# Autodesk Inventor assembly: comp convey
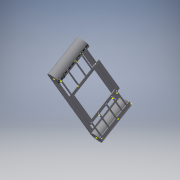
[picture p0: Inventor's stored thumbnail of the model, 180x180]
Saved by Autodesk Inventor 2019 (Build 230136000, 136)
## iProperties
Created: 2020-02-27
Part Number: comp convey
Document SubType Name: Assembly
Designer: LENOVO
Author: LENOVO
## Documents named in this file (5)
- C:\Users\LENOVO\Desktop\Abhishek\comp convey.iam
- C:\Users\LENOVO\Desktop\Abhishek\conv.ipt
- C:\Users\LENOVO\Desktop\Abhishek\connector rod.ipt
- C:\Users\LENOVO\Desktop\Abhishek\connector.ipt
- C:\Users\LENOVO\Desktop\Abhishek\roll.ipt
## Components (34 placed, 4 different names)
1. conv:1 — Mate:3, Mate:8, Mate:11, Mate:14, Mate:15, Mate:17, Mate:18, Mate:19, Mate:24, Mate:25, Mate:30, Mate:31, Mate:36, Mate:37, Mate:38, Mate:39, Mate:40, Mate:49, Mate:50, Mate:51, Mate:52, Mate:53, Mate:54, Mate:55, Mate:56, Mate:57, Mate:58, Mate:59, Mate:60, Mate:61, Mate:62, Mate:63, Mate:64, Mate:65, Mate:66, Mate:81, Mate:83, Mate:84, Mate:85, Mate:86
2. connector rod:1 — Mate:18, Mate:19, Mate:20, Mate:21, Mate:22, Mate:23
3. connector rod:2 — Mate:11, Mate:12, Mate:13, Mate:16
4. connector rod:3 — Mate:24, Mate:25, Mate:26, Mate:27, Mate:28, Mate:29
5. connector rod:5 — Mate:2, Mate:4, Mate:5, Mate:6, Mate:7, Mate:9, Mate:10
6. connector rod:6 — Mate:70, Mate:71, Mate:79
7. connector rod:7 — Mate:72, Mate:73, Mate:77
8. connector rod:8 — Mate:69, Mate:78, Mate:82
9. connector rod:10 — Mate:30, Mate:31, Mate:32, Mate:33, Mate:34, Mate:35
10. connector:1 — Mate:6, Mate:7
11. connector:3 — Mate:9, Mate:10, Mate:17
12. connector:4 — Mate:12, Mate:13, Mate:14
13. connector:7 — Mate:15, Mate:16
14. connector:8 — Mate:26, Mate:29
15. connector:9 — Mate:22, Mate:23
16. connector:10 — Mate:20, Mate:21, Mate:38
17. connector:11 — Mate:2, Mate:3, Mate:4, Mate:5, Mate:8
18. connector:12 — Mate:27, Mate:28, Mate:37
19. connector:14 — Mate:65, Mate:66, Mate:69, Mate:78
20. connector:15 — Mate:34, Mate:35, Mate:36
21. connector:16 — Mate:32, Mate:33
22. connector:17 — Mate:51, Mate:52, Mate:67
23. connector:18 — Mate:53, Mate:54, Mate:70, Mate:79
24. connector:19 — Mate:49, Mate:50
25. connector:20 — Mate:55, Mate:56, Mate:71
26. connector rod:11 — Mate:39, Mate:40, Mate:67
27. connector:21 — Mate:57, Mate:58, Mate:73
28. connector:22 — Mate:63, Mate:64, Mate:72, Mate:77
29. connector:24 — Mate:61, Mate:62, Mate:74
30. connector:25 — Mate:59, Mate:60, Mate:75, Mate:76
31. connector rod:12 — Mate:74, Mate:75, Mate:76
32. connector:26 — Mate:81, Mate:82
33. roll:1 — Mate:83, Mate:84
34. roll:2 — Mate:85, Mate:86
## Relationships (75: Mate 75)
- Mate:2: connector rod:5 ↔ connector:11
- Mate:3: conv:1 ↔ connector:11
- Mate:4: connector rod:5 ↔ connector:11
- Mate:5: connector rod:5 ↔ connector:11
- Mate:6: connector rod:5 ↔ connector:1
- Mate:7: connector rod:5 ↔ connector:1
- Mate:8: conv:1 ↔ connector:11
- Mate:9: connector rod:5 ↔ connector:3
- Mate:10: connector rod:5 ↔ connector:3
- Mate:11: conv:1 ↔ connector rod:2
- Mate:12: connector rod:2 ↔ connector:4
- Mate:13: connector rod:2 ↔ connector:4
- Mate:14: conv:1 ↔ connector:4
- Mate:15: conv:1 ↔ connector:7
- Mate:16: connector rod:2 ↔ connector:7
- Mate:17: conv:1 ↔ connector:3
- Mate:18: conv:1 ↔ connector rod:1
- Mate:19: conv:1 ↔ connector rod:1
- Mate:20: connector rod:1 ↔ connector:10
- Mate:21: connector rod:1 ↔ connector:10
- Mate:22: connector rod:1 ↔ connector:9
- Mate:23: connector rod:1 ↔ connector:9
- Mate:24: conv:1 ↔ connector rod:3
- Mate:25: conv:1 ↔ connector rod:3
- Mate:26: connector rod:3 ↔ connector:8
- Mate:27: connector rod:3 ↔ connector:12
- Mate:28: connector rod:3 ↔ connector:12
- Mate:29: connector rod:3 ↔ connector:8
- Mate:30: conv:1 ↔ connector rod:10
- Mate:31: conv:1 ↔ connector rod:10
- Mate:32: connector rod:10 ↔ connector:16
- Mate:33: connector rod:10 ↔ connector:16
- Mate:34: connector rod:10 ↔ connector:15
- Mate:35: connector rod:10 ↔ connector:15
- Mate:36: conv:1 ↔ connector:15
- Mate:37: conv:1 ↔ connector:12
- Mate:38: conv:1 ↔ connector:10
- Mate:39: conv:1 ↔ connector rod:11
- Mate:40: conv:1 ↔ connector rod:11
- Mate:49: conv:1 ↔ connector:19
- Mate:50: conv:1 ↔ connector:19
- Mate:51: conv:1 ↔ connector:17
- Mate:52: conv:1 ↔ connector:17
- Mate:53: conv:1 ↔ connector:18
- Mate:54: conv:1 ↔ connector:18
- Mate:55: conv:1 ↔ connector:20
- Mate:56: conv:1 ↔ connector:20
- Mate:57: conv:1 ↔ connector:21
- Mate:58: conv:1 ↔ connector:21
- Mate:59: conv:1 ↔ connector:25
- Mate:60: conv:1 ↔ connector:25
- Mate:61: conv:1 ↔ connector:24
- Mate:62: conv:1 ↔ connector:24
- Mate:63: conv:1 ↔ connector:22
- Mate:64: conv:1 ↔ connector:22
- Mate:65: conv:1 ↔ connector:14
- Mate:66: conv:1 ↔ connector:14
- Mate:67: connector:17 ↔ connector rod:11
- Mate:69: connector rod:8 ↔ connector:14
- Mate:70: connector rod:6 ↔ connector:18
- Mate:71: connector rod:6 ↔ connector:20
- Mate:72: connector rod:7 ↔ connector:22
- Mate:73: connector rod:7 ↔ connector:21
- Mate:74: connector:24 ↔ connector rod:12
- Mate:75: connector:25 ↔ connector rod:12
- Mate:76: connector:25 ↔ connector rod:12
- Mate:77: connector rod:7 ↔ connector:22
- Mate:78: connector rod:8 ↔ connector:14
- Mate:79: connector rod:6 ↔ connector:18
- Mate:81: conv:1 ↔ connector:26
- Mate:82: connector rod:8 ↔ connector:26
- Mate:83: conv:1 ↔ roll:1
- Mate:84: conv:1 ↔ roll:1
- Mate:85: conv:1 ↔ roll:2
- Mate:86: conv:1 ↔ roll:2
